# Autodesk Inventor assembly: TourniquetPCBV1_Updated
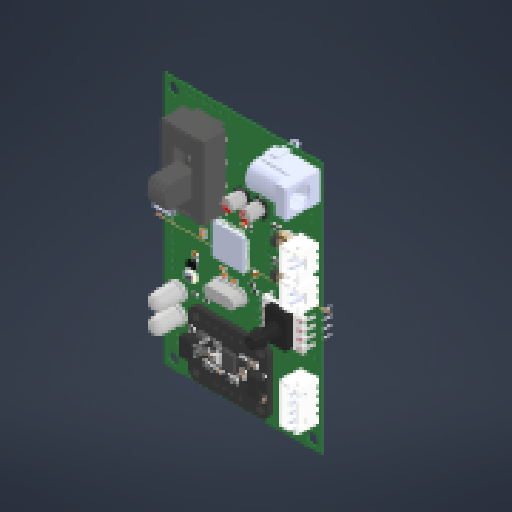
[picture p0: Inventor's stored thumbnail of the model, 512x512]
Saved by Autodesk Inventor 2026.2 (Build 302298000, 298)
## iProperties
Company: Open CASCADE
Created: 2026-02-03
Part Number: TourniquetPCBV1_Updated
Description: Open CASCADE Model
Document SubType Name: Assembly
Designer: vckot
Authority: Unknown
Sending System: Open CASCADE 7.5
Preprocessor: Open CASCADE STEP processor 7.5
Title: Open CASCADE Shape Model
Author: Author
## Documents named in this file (52)
- C:\Users\vckot\OneDrive\Documents\Vaibhav\capstone\CAD_files\PCB\TourniquetPCBV1_Updated\TourniquetPCBV1_Updated\TourniquetPCBV1_Updated.iam
- C:\Users\vckot\OneDrive\Documents\Vaibhav\capstone\CAD_files\PCB\TourniquetPCBV1_Updated\TourniquetPCBV1_Updated\Board.iam
- C:\Users\vckot\OneDrive\Documents\Vaibhav\capstone\CAD_files\PCB\TourniquetPCBV1_Updated\TourniquetPCBV1_Updated\SW2.iam
- C:\Users\vckot\OneDrive\Documents\Vaibhav\capstone\CAD_files\PCB\TourniquetPCBV1_Updated\TourniquetPCBV1_Updated\C16.iam
- C:\Users\vckot\OneDrive\Documents\Vaibhav\capstone\CAD_files\PCB\TourniquetPCBV1_Updated\TourniquetPCBV1_Updated\D7.iam
- C:\Users\vckot\OneDrive\Documents\Vaibhav\capstone\CAD_files\PCB\TourniquetPCBV1_Updated\TourniquetPCBV1_Updated\U5.iam
- C:\Users\vckot\OneDrive\Documents\Vaibhav\capstone\CAD_files\PCB\TourniquetPCBV1_Updated\TourniquetPCBV1_Updated\R21.iam
- C:\Users\vckot\OneDrive\Documents\Vaibhav\capstone\CAD_files\PCB\TourniquetPCBV1_Updated\TourniquetPCBV1_Updated\R20.iam
- C:\Users\vckot\OneDrive\Documents\Vaibhav\capstone\CAD_files\PCB\TourniquetPCBV1_Updated\TourniquetPCBV1_Updated\R19.iam
- C:\Users\vckot\OneDrive\Documents\Vaibhav\capstone\CAD_files\PCB\TourniquetPCBV1_Updated\TourniquetPCBV1_Updated\R2.iam
- C:\Users\vckot\OneDrive\Documents\Vaibhav\capstone\CAD_files\PCB\TourniquetPCBV1_Updated\TourniquetPCBV1_Updated\J6.iam
- C:\Users\vckot\OneDrive\Documents\Vaibhav\capstone\CAD_files\PCB\TourniquetPCBV1_Updated\TourniquetPCBV1_Updated\J5.iam
- C:\Users\vckot\OneDrive\Documents\Vaibhav\capstone\CAD_files\PCB\TourniquetPCBV1_Updated\TourniquetPCBV1_Updated\R9.iam
- C:\Users\vckot\OneDrive\Documents\Vaibhav\capstone\CAD_files\PCB\TourniquetPCBV1_Updated\TourniquetPCBV1_Updated\R7.iam
- C:\Users\vckot\OneDrive\Documents\Vaibhav\capstone\CAD_files\PCB\TourniquetPCBV1_Updated\TourniquetPCBV1_Updated\R5.iam
- C:\Users\vckot\OneDrive\Documents\Vaibhav\capstone\CAD_files\PCB\TourniquetPCBV1_Updated\TourniquetPCBV1_Updated\R3.iam
- C:\Users\vckot\OneDrive\Documents\Vaibhav\capstone\CAD_files\PCB\TourniquetPCBV1_Updated\TourniquetPCBV1_Updated\R11.iam
- C:\Users\vckot\OneDrive\Documents\Vaibhav\capstone\CAD_files\PCB\TourniquetPCBV1_Updated\TourniquetPCBV1_Updated\R10.iam
- C:\Users\vckot\OneDrive\Documents\Vaibhav\capstone\CAD_files\PCB\TourniquetPCBV1_Updated\TourniquetPCBV1_Updated\U4.iam
- C:\Users\vckot\OneDrive\Documents\Vaibhav\capstone\CAD_files\PCB\TourniquetPCBV1_Updated\TourniquetPCBV1_Updated\U1.iam
- C:\Users\vckot\OneDrive\Documents\Vaibhav\capstone\CAD_files\PCB\TourniquetPCBV1_Updated\TourniquetPCBV1_Updated\SW1.iam
- C:\Users\vckot\OneDrive\Documents\Vaibhav\capstone\CAD_files\PCB\TourniquetPCBV1_Updated\TourniquetPCBV1_Updated\R16.iam
- C:\Users\vckot\OneDrive\Documents\Vaibhav\capstone\CAD_files\PCB\TourniquetPCBV1_Updated\TourniquetPCBV1_Updated\R15.iam
- C:\Users\vckot\OneDrive\Documents\Vaibhav\capstone\CAD_files\PCB\TourniquetPCBV1_Updated\TourniquetPCBV1_Updated\R14.iam
- C:\Users\vckot\OneDrive\Documents\Vaibhav\capstone\CAD_files\PCB\TourniquetPCBV1_Updated\TourniquetPCBV1_Updated\R13.iam
- C:\Users\vckot\OneDrive\Documents\Vaibhav\capstone\CAD_files\PCB\TourniquetPCBV1_Updated\TourniquetPCBV1_Updated\R12.iam
- C:\Users\vckot\OneDrive\Documents\Vaibhav\capstone\CAD_files\PCB\TourniquetPCBV1_Updated\TourniquetPCBV1_Updated\R6.iam
- C:\Users\vckot\OneDrive\Documents\Vaibhav\capstone\CAD_files\PCB\TourniquetPCBV1_Updated\TourniquetPCBV1_Updated\R1.iam
- C:\Users\vckot\OneDrive\Documents\Vaibhav\capstone\CAD_files\PCB\TourniquetPCBV1_Updated\TourniquetPCBV1_Updated\Q3.iam
- C:\Users\vckot\OneDrive\Documents\Vaibhav\capstone\CAD_files\PCB\TourniquetPCBV1_Updated\TourniquetPCBV1_Updated\Q1.iam
- C:\Users\vckot\OneDrive\Documents\Vaibhav\capstone\CAD_files\PCB\TourniquetPCBV1_Updated\TourniquetPCBV1_Updated\O1.iam
- C:\Users\vckot\OneDrive\Documents\Vaibhav\capstone\CAD_files\PCB\TourniquetPCBV1_Updated\TourniquetPCBV1_Updated\J3.iam
- C:\Users\vckot\OneDrive\Documents\Vaibhav\capstone\CAD_files\PCB\TourniquetPCBV1_Updated\TourniquetPCBV1_Updated\J1.iam
- C:\Users\vckot\OneDrive\Documents\Vaibhav\capstone\CAD_files\PCB\TourniquetPCBV1_Updated\TourniquetPCBV1_Updated\FB1.iam
- C:\Users\vckot\OneDrive\Documents\Vaibhav\capstone\CAD_files\PCB\TourniquetPCBV1_Updated\TourniquetPCBV1_Updated\D5.iam
- C:\Users\vckot\OneDrive\Documents\Vaibhav\capstone\CAD_files\PCB\TourniquetPCBV1_Updated\TourniquetPCBV1_Updated\D4.iam
- C:\Users\vckot\OneDrive\Documents\Vaibhav\capstone\CAD_files\PCB\TourniquetPCBV1_Updated\TourniquetPCBV1_Updated\D3.iam
- C:\Users\vckot\OneDrive\Documents\Vaibhav\capstone\CAD_files\PCB\TourniquetPCBV1_Updated\TourniquetPCBV1_Updated\D1.iam
- C:\Users\vckot\OneDrive\Documents\Vaibhav\capstone\CAD_files\PCB\TourniquetPCBV1_Updated\TourniquetPCBV1_Updated\C15.iam
- C:\Users\vckot\OneDrive\Documents\Vaibhav\capstone\CAD_files\PCB\TourniquetPCBV1_Updated\TourniquetPCBV1_Updated\C12.iam
- C:\Users\vckot\OneDrive\Documents\Vaibhav\capstone\CAD_files\PCB\TourniquetPCBV1_Updated\TourniquetPCBV1_Updated\C11.iam
- C:\Users\vckot\OneDrive\Documents\Vaibhav\capstone\CAD_files\PCB\TourniquetPCBV1_Updated\TourniquetPCBV1_Updated\C10.iam
- C:\Users\vckot\OneDrive\Documents\Vaibhav\capstone\CAD_files\PCB\TourniquetPCBV1_Updated\TourniquetPCBV1_Updated\C9.iam
- C:\Users\vckot\OneDrive\Documents\Vaibhav\capstone\CAD_files\PCB\TourniquetPCBV1_Updated\TourniquetPCBV1_Updated\C8.iam
- C:\Users\vckot\OneDrive\Documents\Vaibhav\capstone\CAD_files\PCB\TourniquetPCBV1_Updated\TourniquetPCBV1_Updated\C7.iam
- C:\Users\vckot\OneDrive\Documents\Vaibhav\capstone\CAD_files\PCB\TourniquetPCBV1_Updated\TourniquetPCBV1_Updated\C6.iam
- C:\Users\vckot\OneDrive\Documents\Vaibhav\capstone\CAD_files\PCB\TourniquetPCBV1_Updated\TourniquetPCBV1_Updated\C5.iam
- C:\Users\vckot\OneDrive\Documents\Vaibhav\capstone\CAD_files\PCB\TourniquetPCBV1_Updated\TourniquetPCBV1_Updated\C4.iam
- C:\Users\vckot\OneDrive\Documents\Vaibhav\capstone\CAD_files\PCB\TourniquetPCBV1_Updated\TourniquetPCBV1_Updated\C3.iam
- C:\Users\vckot\OneDrive\Documents\Vaibhav\capstone\CAD_files\PCB\TourniquetPCBV1_Updated\TourniquetPCBV1_Updated\C2.iam
- C:\Users\vckot\OneDrive\Documents\Vaibhav\capstone\CAD_files\PCB\TourniquetPCBV1_Updated\TourniquetPCBV1_Updated\C1.iam
- C:\Users\vckot\OneDrive\Documents\Vaibhav\capstone\CAD_files\PCB\TourniquetPCBV1_Updated\TourniquetPCBV1_Updated\_.iam
## Components (51 placed, 51 different names)
1. Board_2 [sub-assembly] — Flush:1
2. SW2_9 [sub-assembly]
3. C16_13 [sub-assembly]
4. D7_18 [sub-assembly]
5. U5_45 [sub-assembly]
6. R21_47 [sub-assembly]
7. R20_49 [sub-assembly]
8. R19_51 [sub-assembly]
9. R2_53 [sub-assembly]
10. J6_56 [sub-assembly]
11. J5_65 [sub-assembly]
12. R9_67 [sub-assembly]
13. R7_69 [sub-assembly]
14. R5_71 [sub-assembly]
15. R3_73 [sub-assembly]
16. R11_75 [sub-assembly]
17. R10_77 [sub-assembly]
18. U4_79 [sub-assembly]
19. U1_81 [sub-assembly]
20. SW1_83 [sub-assembly]
21. R16_85 [sub-assembly]
22. R15_87 [sub-assembly]
23. R14_89 [sub-assembly]
24. R13_91 [sub-assembly]
25. R12_93 [sub-assembly]
26. R6_95 [sub-assembly]
27. R1_97 [sub-assembly]
28. Q3_99 [sub-assembly]
29. Q1_101 [sub-assembly]
30. O1_103 [sub-assembly]
31. J3_106 [sub-assembly]
32. J1_108 [sub-assembly]
33. FB1_113 [sub-assembly]
34. D5_115 [sub-assembly]
35. D4_117 [sub-assembly]
36. D3_119 [sub-assembly]
37. D1_121 [sub-assembly]
38. C15_123 [sub-assembly]
39. C12_125 [sub-assembly]
40. C11_127 [sub-assembly]
41. C10_129 [sub-assembly]
42. C9_131 [sub-assembly]
43. C8_133 [sub-assembly]
44. C7_135 [sub-assembly]
45. C6_137 [sub-assembly]
46. C5_139 [sub-assembly]
47. C4_141 [sub-assembly]
48. C3_143 [sub-assembly]
49. C2_145 [sub-assembly]
50. C1_147 [sub-assembly]
51. __149 [sub-assembly]
## Relationships (1: Flush 1)
- Flush:1 (-40 mm): Board_2
